# Autodesk Inventor assembly: コガネイシリンダMBDA615
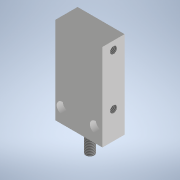
[picture p0: Inventor's stored thumbnail of the model, 180x180]
Saved by Autodesk Inventor 2021 (Build 250183000, 183)
## iProperties
Created: 2021-09-24
Part Number: コガネイシリンダMBDA615
Document SubType Name: Assembly
Designer: tomat
Author: tomat
## Documents named in this file (4)
- C:\Users\ryusei\Documents\Inventor\robot_design3\試作品1号\MBDA6×15_シリンダコガネイ\コガネイシリンダMBDA615.iam
- C:\Users\ryusei\Documents\Inventor\robot_design3\試作品1号\MBDA6×15_シリンダコガネイ\本体.ipt
- C:\Users\ryusei\Documents\Inventor\robot_design3\試作品1号\MBDA6×15_シリンダコガネイ\伸びるやつ１.ipt
- C:\Users\ryusei\Documents\Inventor\robot_design3\試作品1号\MBDA6×15_シリンダコガネイ\伸びるやつ2.ipt
## Components (3 placed, 3 different names)
1. 本体:1 — 円柱状:1
2. 伸びるやつ１:1 — 挿入:1, 円柱状:1
3. 伸びるやつ2:1 — 挿入:1
## Relationships (2: Insert 1, CylindricalJoint 1)
- 挿入:1 [Insert]: 伸びるやつ１:1 ↔ 伸びるやつ2:1
- 円柱状:1 [CylindricalJoint]: 本体:1 ↔ 伸びるやつ１:1
